# Autodesk Inventor assembly: 棒球工板組合
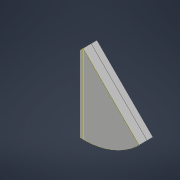
[picture p0: Inventor's stored thumbnail of the model, 180x180]
Saved by Autodesk Inventor 2021 (Build 250183000, 183)
## iProperties
Created: 2020-12-24
Part Number: 棒球工板組合
Document SubType Name: Assembly
Designer: zihon
Author: zihon
## Documents named in this file (4)
- C:\Users\zihon\Desktop\棒球公版\棒球組合 - 公版.iam
- C:\Users\zihon\Desktop\棒球公版\球場2 - 公版.ipt
- C:\Users\zihon\Desktop\棒球公版\棒球底座 - 公版.ipt
- C:\Users\zihon\Downloads\球棒.ipt
## Components (3 placed, 3 different names)
1. 球場2 - 公版:1 — 貼合:1, 貼合:2, 角度:1, 貼合:3, 貼合:4, 貼合:5, 貼合:6, 相切:1, 貼合:7
2. 棒球底座 - 公版:1 — 貼合:4, 貼合:5, 貼合:6
3. 球棒:1 — 相切:1, 貼合:7
## Relationships (9: Mate 7, Angle 1, Tangent 1)
- 貼合:1 [Mate]: 球場2 - 公版:1
- 貼合:2 [Mate]: 球場2 - 公版:1
- 角度:1 [Angle] (45 deg): 球場2 - 公版:1
- 貼合:3 [Mate]: 球場2 - 公版:1
- 貼合:4 [Mate]: 球場2 - 公版:1 ↔ 棒球底座 - 公版:1
- 貼合:5 [Mate]: 球場2 - 公版:1 ↔ 棒球底座 - 公版:1
- 貼合:6 [Mate]: 球場2 - 公版:1 ↔ 棒球底座 - 公版:1
- 相切:1 [Tangent]: 球場2 - 公版:1 ↔ 球棒:1
- 貼合:7 [Mate]: 球場2 - 公版:1 ↔ 球棒:1
